# Autodesk Inventor assembly: 3 mm
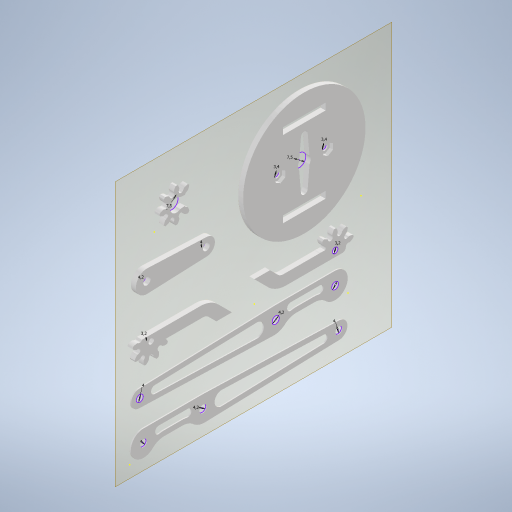
[picture p0: Inventor's stored thumbnail of the model, 512x512]
Saved by Autodesk Inventor 2023 (Build 270158000, 158)
## iProperties
Created: 2023-11-09
Part Number: 3 mm
Document SubType Name: Assembly
Designer: JULIAN
Author: JULIAN
## Documents named in this file (7)
- C:\Users\JULIAN\Desktop\Materias UN\Taller de Ingeniería Electrónica\Modelado cargo bot\DXF\3 mm.iam
- C:\Users\JULIAN\Desktop\Materias UN\Taller de Ingeniería Electrónica\Modelado cargo bot\Modelado\Brazo conductor vertical.ipt
- C:\Users\JULIAN\Desktop\Materias UN\Taller de Ingeniería Electrónica\Modelado cargo bot\Modelado\Brazo engrane 2.ipt
- C:\Users\JULIAN\Desktop\Materias UN\Taller de Ingeniería Electrónica\Modelado cargo bot\Modelado\Brazo engrane.ipt
- C:\Users\JULIAN\Desktop\Materias UN\Taller de Ingeniería Electrónica\Modelado cargo bot\Modelado\Engrane.ipt
- C:\Users\JULIAN\Desktop\Materias UN\Taller de Ingeniería Electrónica\Modelado cargo bot\Modelado\Plato base.ipt
- C:\Users\JULIAN\Desktop\Materias UN\Taller de Ingeniería Electrónica\Modelado cargo bot\Modelado\Brazo horizontal 2.ipt
## Components (7 placed, 6 different names)
1. Brazo conductor vertical:1 — Coincidencia:7
2. Brazo engrane 2:1 — Coincidencia:3
3. Brazo engrane:1 — Coincidencia:4
4. Engrane:1 — Coincidencia:6
5. Plato base:1 — Coincidencia:5
6. Brazo horizontal 2:1 — Coincidencia:8
7. Brazo horizontal 2:2 — Coincidencia:1
## Relationships (7: Mate 7)
- Coincidencia:1 [Mate]: Brazo horizontal 2:2
- Coincidencia:3 [Mate]: Brazo engrane 2:1
- Coincidencia:4 [Mate]: Brazo engrane:1
- Coincidencia:5 [Mate]: Plato base:1
- Coincidencia:6 [Mate]: Engrane:1
- Coincidencia:7 [Mate]: Brazo conductor vertical:1
- Coincidencia:8 [Mate]: Brazo horizontal 2:1
